# Autodesk Inventor assembly: TestFixture
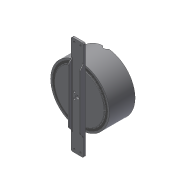
[picture p0: Inventor's stored thumbnail of the model, 180x180]
Saved by Autodesk Inventor 2018 (Build 220112000, 112)
## iProperties
Created: 2019-09-26
Part Number: TestFixture
Document SubType Name: Assembly
Designer: Clevo
Author: Clevo
## Documents named in this file (5)
- E:\RobotArm\MCAD\TestFixture\TestFixture.iam
- E:\RobotArm\MCAD\TestFixture\TestBase.ipt
- E:\RobotArm\MCAD\LX-16A.iam
- E:\RobotArm\MCAD\TestFixture\IndPlate.ipt
- E:\RobotArm\MCAD\TestFixture\TestArm.ipt
## Components (4 placed, 4 different names)
1. TestBase:1 — Mate:1, Mate:2, Angle:1
2. LX-16A:1 [sub-assembly] — Mate:1, Mate:2, Angle:1, Mate:3, Mate:4, Mate:5
3. IndPlate:1 — Mate:3, Mate:4, Mate:5, Mate:6, Mate:7, Mate:8
4. TestArm:1 — Mate:6, Mate:7, Mate:8
## Relationships (9: Mate 8, Angle 1)
- Mate:1: TestBase:1 ↔ LX-16A:1
- Mate:2: TestBase:1 ↔ LX-16A:1
- Angle:1 (90 deg): TestBase:1 ↔ LX-16A:1
- Mate:3: LX-16A:1 ↔ IndPlate:1
- Mate:4: LX-16A:1 ↔ IndPlate:1
- Mate:5: LX-16A:1 ↔ IndPlate:1
- Mate:6: IndPlate:1 ↔ TestArm:1
- Mate:7: IndPlate:1 ↔ TestArm:1
- Mate:8: IndPlate:1 ↔ TestArm:1
